# Autodesk Inventor assembly: Stewart-Base-KST-DS215
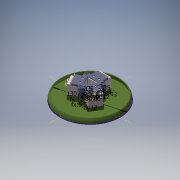
[picture p0: Inventor's stored thumbnail of the model, 180x180]
Saved by Autodesk Inventor 2018.2 (Build 222227000, 227)
## iProperties
Created: 2018-02-24
Part Number: Stewart-Base-KST-DS215
Material: Generisch
Document SubType Name: Assembly
Designer: JochenAlt
Author: JochenAlt
## Documents named in this file (3)
- D:\Projects\Donna\CAD\KST DS215MG\Stewart-Base-KST-DS215.iam
- D:\Projects\Donna\CAD\KST DS215MG\Stewart-Platform-Base-KST-DS215MG.ipt
- D:\Projects\Donna\CAD\KST DS215MG\Servo-KST-DS215MG.ipt
## Components (7 placed, 2 different names)
1. Stewart-Platform-Base-KST-DS215MG:1 — Passend:3, Passend:4, Passend:34, Passend:35, Passend:36, Passend:37, Passend:38, Passend:39, Passend:40, Passend:41, Passend:42, Passend:43, Passend:44, Passend:45, Passend:46, Passend:47, Passend:48, Passend:49, Passend:50, Passend:51, Passend:52, Passend:53, Passend:54
2. Servo-KST-DS215MG:1 — Passend:36, Passend:38, Passend:40, Passend:41
3. Servo-KST-DS215MG:2 — Passend:37, Passend:39, Passend:42
4. Servo-KST-DS215MG:3 — Passend:43, Passend:45, Passend:47
5. Servo-KST-DS215MG:4 — Passend:44, Passend:46, Passend:48
6. Servo-KST-DS215MG:5 — Passend:49, Passend:51, Passend:54
7. Servo-KST-DS215MG:6 — Passend:50, Passend:52, Passend:53
## Relationships (23: Mate 23)
- Passend:3 [Mate]: Stewart-Platform-Base-KST-DS215MG:1
- Passend:4 [Mate]: Stewart-Platform-Base-KST-DS215MG:1
- Passend:34 [Mate]: Stewart-Platform-Base-KST-DS215MG:1
- Passend:35 [Mate]: Stewart-Platform-Base-KST-DS215MG:1
- Passend:36 [Mate]: Stewart-Platform-Base-KST-DS215MG:1 ↔ Servo-KST-DS215MG:1
- Passend:37 [Mate]: Stewart-Platform-Base-KST-DS215MG:1 ↔ Servo-KST-DS215MG:2
- Passend:38 [Mate]: Stewart-Platform-Base-KST-DS215MG:1 ↔ Servo-KST-DS215MG:1
- Passend:39 [Mate]: Stewart-Platform-Base-KST-DS215MG:1 ↔ Servo-KST-DS215MG:2
- Passend:40 [Mate]: Stewart-Platform-Base-KST-DS215MG:1 ↔ Servo-KST-DS215MG:1
- Passend:41 [Mate]: Stewart-Platform-Base-KST-DS215MG:1 ↔ Servo-KST-DS215MG:1
- Passend:42 [Mate]: Stewart-Platform-Base-KST-DS215MG:1 ↔ Servo-KST-DS215MG:2
- Passend:43 [Mate]: Stewart-Platform-Base-KST-DS215MG:1 ↔ Servo-KST-DS215MG:3
- Passend:44 [Mate]: Stewart-Platform-Base-KST-DS215MG:1 ↔ Servo-KST-DS215MG:4
- Passend:45 [Mate]: Stewart-Platform-Base-KST-DS215MG:1 ↔ Servo-KST-DS215MG:3
- Passend:46 [Mate]: Stewart-Platform-Base-KST-DS215MG:1 ↔ Servo-KST-DS215MG:4
- Passend:47 [Mate]: Stewart-Platform-Base-KST-DS215MG:1 ↔ Servo-KST-DS215MG:3
- Passend:48 [Mate]: Stewart-Platform-Base-KST-DS215MG:1 ↔ Servo-KST-DS215MG:4
- Passend:49 [Mate]: Stewart-Platform-Base-KST-DS215MG:1 ↔ Servo-KST-DS215MG:5
- Passend:50 [Mate]: Stewart-Platform-Base-KST-DS215MG:1 ↔ Servo-KST-DS215MG:6
- Passend:51 [Mate]: Stewart-Platform-Base-KST-DS215MG:1 ↔ Servo-KST-DS215MG:5
- Passend:52 [Mate]: Stewart-Platform-Base-KST-DS215MG:1 ↔ Servo-KST-DS215MG:6
- Passend:53 [Mate]: Stewart-Platform-Base-KST-DS215MG:1 ↔ Servo-KST-DS215MG:6
- Passend:54 [Mate]: Stewart-Platform-Base-KST-DS215MG:1 ↔ Servo-KST-DS215MG:5
